# Autodesk Inventor assembly: 742a 2.1 Intake Carriage
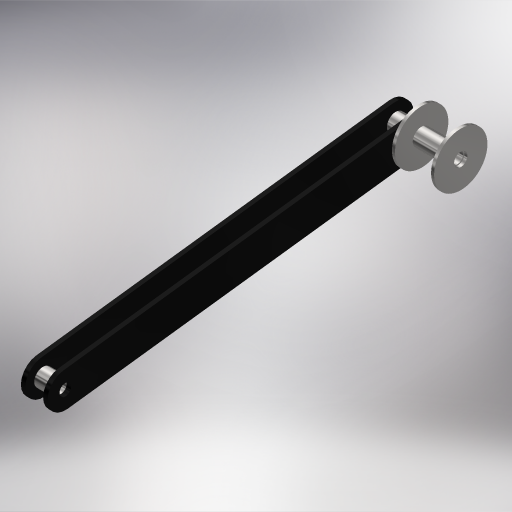
[picture p0: Inventor's stored thumbnail of the model, 512x512]
Saved by Autodesk Inventor 2024 (Build 280153000, 153)
## iProperties
Created: 2023-10-21
Part Number: 742a 2.1 Intake Carriage
Document SubType Name: Assembly
Designer: aaron
Author: aaron
## Documents named in this file (4)
- C:\Users\aaron\Documents\Inventor\TritonRobotics\library\Subsystems\742a 2.1 Intake Carriage.iam
- C:\Users\aaron\Documents\Inventor\TritonRobotics\library\Stock Material\Plates New\Intake Carriage.ipt
- C:\Users\aaron\Documents\Inventor\TritonRobotics\library\VEX Library\Structure\Metal Spacers\0.25 1-2 od.ipt
- C:\Users\aaron\Documents\Inventor\TritonRobotics\library\VEX Library\Motion\Spacers\0.75 od spcaer.ipt
## Components (8 placed, 3 different names)
1. Intake Carriage:1 — Mate:5, Mate:6, Mate:7, Mate:8, Mate:9
2. Intake Carriage:2 — Mate:1, Mate:2, Mate:3, Mate:4
3. 0.25 1-2 od:1 — Mate:1, Mate:2, Mate:7
4. 0.25 1-2 od:2 — Mate:3, Mate:4, Mate:5, Mate:6
5. 0.75 od spcaer:1 — Mate:8, Mate:9, Mate:12, Mate:13
6. 0.25 1-2 od:3 — Mate:10, Mate:11, Mate:12, Mate:13
7. 0.25 1-2 od:4 — Mate:10, Mate:11, Mate:14, Mate:15
8. 0.75 od spcaer:2 — Mate:14, Mate:15
## Relationships (15: Mate 15)
- Mate:1: Intake Carriage:2 ↔ 0.25 1-2 od:1
- Mate:2: Intake Carriage:2 ↔ 0.25 1-2 od:1
- Mate:3: Intake Carriage:2 ↔ 0.25 1-2 od:2
- Mate:4: Intake Carriage:2 ↔ 0.25 1-2 od:2
- Mate:5: Intake Carriage:1 ↔ 0.25 1-2 od:2
- Mate:6: Intake Carriage:1 ↔ 0.25 1-2 od:2
- Mate:7: Intake Carriage:1 ↔ 0.25 1-2 od:1
- Mate:8: Intake Carriage:1 ↔ 0.75 od spcaer:1
- Mate:9: Intake Carriage:1 ↔ 0.75 od spcaer:1
- Mate:10: 0.25 1-2 od:3 ↔ 0.25 1-2 od:4
- Mate:11: 0.25 1-2 od:3 ↔ 0.25 1-2 od:4
- Mate:12: 0.75 od spcaer:1 ↔ 0.25 1-2 od:3
- Mate:13: 0.75 od spcaer:1 ↔ 0.25 1-2 od:3
- Mate:14: 0.25 1-2 od:4 ↔ 0.75 od spcaer:2
- Mate:15: 0.25 1-2 od:4 ↔ 0.75 od spcaer:2
